# Autodesk Inventor assembly: SmallSkirtWall
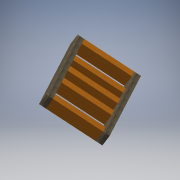
[picture p0: Inventor's stored thumbnail of the model, 180x180]
Saved by Autodesk Inventor 2016 (Build 200138000, 138)
## iProperties
Created: 2016-06-15
Part Number: SmallSkirtWall
Document SubType Name: Assembly
Designer: cutrones
Author: cutrones
## Documents named in this file (3)
- C:\Users\cutrones\Desktop\MotionBase\CAD\MotionBaseCAD\BaseSkirt\SmallSkirtWall.iam
- C:\Users\cutrones\Desktop\MotionBase\CAD\MotionBaseCAD\BaseSkirt\VertBeam.ipt
- C:\Users\cutrones\Desktop\MotionBase\CAD\MotionBaseCAD\BaseSkirt\SmallHorizBeam.ipt
## Components (7 placed, 2 different names)
1. VertBeam:1 — Mate:2, Flush:3, Flush:4, Flush:5, Flush:6, Mate:4, Mate:10
2. VertBeam:2 — Mate:7, Flush:9, Mate:9
3. VertBeam:3 — Mate:1, Flush:1, Flush:2, Mate:3, Mate:8, Mate:9
4. VertBeam:4 — Mate:6, Flush:8, Mate:8
5. VertBeam:5 — Mate:5, Flush:7, Mate:10
6. SmallHorizBeam:1 — Flush:5, Flush:6, Mate:3, Mate:4
7. SmallHorizBeam:2 — Mate:1, Flush:1, Flush:2, Mate:2, Flush:3, Flush:4, Mate:5, Mate:6, Mate:7, Flush:7, Flush:8, Flush:9
## Relationships (19: Mate 10, Flush 9)
- Mate:1: VertBeam:3 ↔ SmallHorizBeam:2
- Flush:1: VertBeam:3 ↔ SmallHorizBeam:2
- Flush:2: VertBeam:3 ↔ SmallHorizBeam:2
- Mate:2: VertBeam:1 ↔ SmallHorizBeam:2
- Flush:3: VertBeam:1 ↔ SmallHorizBeam:2
- Flush:4: VertBeam:1 ↔ SmallHorizBeam:2
- Flush:5: VertBeam:1 ↔ SmallHorizBeam:1
- Flush:6: VertBeam:1 ↔ SmallHorizBeam:1
- Mate:3: VertBeam:3 ↔ SmallHorizBeam:1
- Mate:4: VertBeam:1 ↔ SmallHorizBeam:1
- Mate:5: VertBeam:5 ↔ SmallHorizBeam:2
- Mate:6: VertBeam:4 ↔ SmallHorizBeam:2
- Mate:7: VertBeam:2 ↔ SmallHorizBeam:2
- Flush:7: VertBeam:5 ↔ SmallHorizBeam:2
- Flush:8: VertBeam:4 ↔ SmallHorizBeam:2
- Flush:9: VertBeam:2 ↔ SmallHorizBeam:2
- Mate:8 (254 mm): VertBeam:3 ↔ VertBeam:4
- Mate:9 (127 mm): VertBeam:2 ↔ VertBeam:3
- Mate:10 (127 mm): VertBeam:1 ↔ VertBeam:5
